# Autodesk Inventor assembly: Thermoelectric Generator
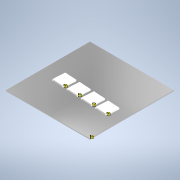
[picture p0: Inventor's stored thumbnail of the model, 180x180]
Saved by Autodesk Inventor 2020 (Build 240168000, 168)
## iProperties
Created: 2021-04-27
Part Number: Thermoelectric Generator
Document SubType Name: Assembly
Designer: User
Author: User
## Documents named in this file (3)
- C:\Users\User\Spring2021\Thermoelectric Generator.iam
- E:\Users\User\Document\Inventor\star design\Conduction Sheet.ipt
- E:\Users\User\Document\Inventor\star design\SP1848-27145 4.8V Seebeck Thermoelectric Power Generator TEG Peltier Module.ipt
## Components (5 placed, 2 different names)
1. Conduction Sheet:1 — Mate:1
2. SP1848-27145 4.8V Seebeck Thermoelectric Power Generator TEG Peltier Module:1 — Mate:1
3. SP1848-27145 4.8V Seebeck Thermoelectric Power Generator TEG Peltier Module:2
4. SP1848-27145 4.8V Seebeck Thermoelectric Power Generator TEG Peltier Module:3
5. SP1848-27145 4.8V Seebeck Thermoelectric Power Generator TEG Peltier Module:4
## Component patterns: (4 elements, first: SP1848-27145 4.8V Seebeck Thermoelectric Power Generator TEG Peltier Module:1)
## Relationships (1: Mate 1)
- Mate:1: Conduction Sheet:1 ↔ SP1848-27145 4.8V Seebeck Thermoelectric Power Generator TEG Peltier Module:1
